# Autodesk Inventor assembly: Pulley
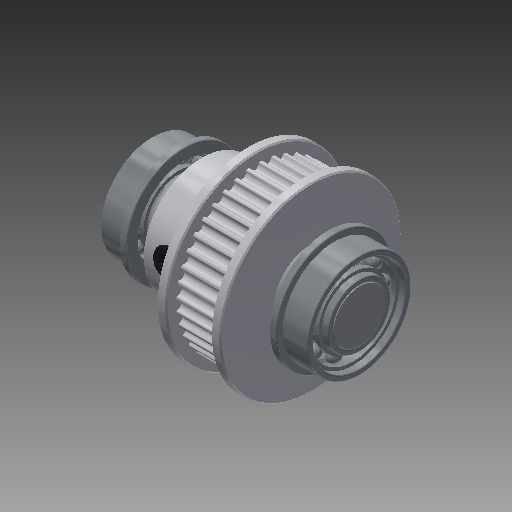
[picture p0: Inventor's stored thumbnail of the model, 512x512]
Saved by Autodesk Inventor 2019.3 (Build 233278000, 278)
## iProperties
Created: 2020-08-25
Part Number: Pulley
Material: Generisch
Document SubType Name: Assembly
Designer: Nicolas Frick
Author: Nicolas Frick
## Documents named in this file (5)
- C:\Users\Nicolas Frick\Sync\OneDrive\airhockeybot\mechanical_design\inventor\Pulley.iam
- C:\Users\Nicolas Frick\Sync\OneDrive\airhockeybot\mechanical_design\inventor\Shaft_8mm.ipt
- C:\Users\Nicolas Frick\Sync\OneDrive\airhockeybot\mechanical_design\inventor\Bearing F688ZZ\F688ZZ_assembly.iam
- C:\Users\Nicolas Frick\Sync\OneDrive\airhockeybot\mechanical_design\inventor\GT2 40T 8mm Bore 6mm wide pulley\GT2 40T 8 Bore v2.iam
- C:\Users\Nicolas Frick\Sync\OneDrive\airhockeybot\mechanical_design\inventor\distance_short.ipt
## Components (6 placed, 4 different names)
1. Shaft_8mm:1 — Drehbar:2, Passend:9, Passend:10, Passend:11, Passend:12, Passend:17
2. F688ZZ_assembly:1 [sub-assembly] — Passend:17, Passend:18
3. F688ZZ_assembly:2 [sub-assembly] — Drehbar:2, Passend:13
4. GT2 40T 8 Bore v2:1 [sub-assembly] — Passend:9, Passend:12, Passend:15, Passend:16
5. distance_short:1 — Passend:10, Passend:13, Passend:15
6. distance_short:2 — Passend:11, Passend:16, Passend:18
## Relationships (10: Mate 9, RevoluteJoint 1)
- Drehbar:2 [RevoluteJoint]: Shaft_8mm:1 ↔ F688ZZ_assembly:2
- Passend:9 [Mate]: Shaft_8mm:1 ↔ GT2 40T 8 Bore v2:1
- Passend:10 [Mate]: Shaft_8mm:1 ↔ distance_short:1
- Passend:11 [Mate]: Shaft_8mm:1 ↔ distance_short:2
- Passend:12 [Mate]: Shaft_8mm:1 ↔ GT2 40T 8 Bore v2:1
- Passend:13 [Mate]: F688ZZ_assembly:2 ↔ distance_short:1
- Passend:15 [Mate]: GT2 40T 8 Bore v2:1 ↔ distance_short:1
- Passend:16 [Mate]: GT2 40T 8 Bore v2:1 ↔ distance_short:2
- Passend:17 [Mate]: Shaft_8mm:1 ↔ F688ZZ_assembly:1
- Passend:18 [Mate]: F688ZZ_assembly:1 ↔ distance_short:2
